# Autodesk Inventor assembly: MIR_HbCircuit
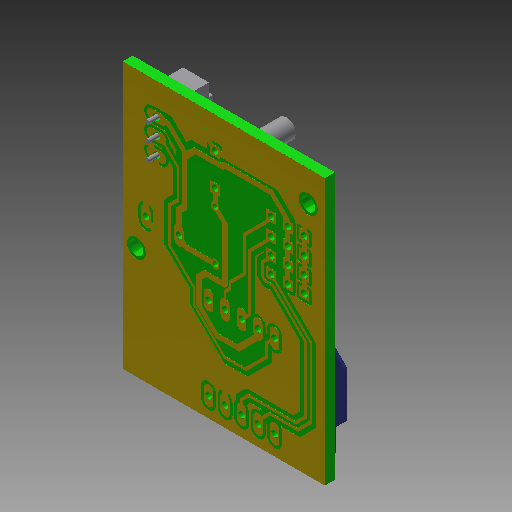
[picture p0: Inventor's stored thumbnail of the model, 512x512]
Saved by Autodesk Inventor 2017 (Build 210142000, 142)
## iProperties
Part Number: MIR_HbCircuit
Material: 一般
Document SubType Name: Assembly
Designer: sktom
Author: sktom
## Documents named in this file (5)
- D:\OneDrive\CAD\MAJ\hackberry\HACKberry-hardware\3D_69%inlength\Inventor\HbHandForChild\HbCircuit\MIR_HbCircuit.iam
- D:\OneDrive\CAD\MAJ\hackberry\HACKberry-hardware\3D_69%inlength\Inventor\HbHandForChild\HbCircuit\MIR_HbSizeS.ipt
- D:\OneDrive\CAD\MAJ\hackberry\HACKberry-hardware\3D_69%inlength\Inventor\HbHandForChild\HbCircuit\MIR_SS-12SDP2.ipt
- D:\OneDrive\CAD\MAJ\hackberry\HACKberry-hardware\3D_69%inlength\Inventor\HbHandForChild\HbCircuit\MIR_trinket 5V.ipt
- D:\OneDrive\CAD\MAJ\hackberry\HACKberry-hardware\3D_69%inlength\Inventor\HbHandForChild\HbCircuit\MIR_SKRGAQD010.ipt
## Components (4 placed, 4 different names)
1. MIR_HbSizeS:1 — 挿入:1, 挿入:3, 挿入:2
2. MIR_SS-12SDP2:1 — 挿入:1
3. MIR_trinket 5V:1 — 挿入:3
4. MIR_SKRGAQD010:1 — 挿入:2
## Relationships (3: Insert 3)
- 挿入:1 [Insert]: MIR_HbSizeS:1 ↔ MIR_SS-12SDP2:1
- 挿入:3 [Insert] (1 mm): MIR_HbSizeS:1 ↔ MIR_trinket 5V:1
- 挿入:2 [Insert]: MIR_HbSizeS:1 ↔ MIR_SKRGAQD010:1
